# Autodesk Inventor assembly: Shooter
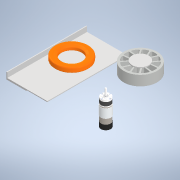
[picture p0: Inventor's stored thumbnail of the model, 180x180]
Saved by Autodesk Inventor 2021 (Build 250183000, 183)
## iProperties
Created: 2020-09-12
Part Number: Shooter
Document SubType Name: Assembly
Designer: deli
Author: deli
## Documents named in this file (7)
- C:\Users\deli\OneDrive - Eastside Preparatory School\FTC\Ultamite Goal\Shooter 9-12-2020.iam
- C:\Users\deli\OneDrive - Eastside Preparatory School\FTC\Ultamite Goal\am-4300 Ring.ipt
- C:\Users\deli\OneDrive - Eastside Preparatory School\FTC\Chassi\Cutting\Drill Patterns\ramp.ipt
- C:\Users\deli\OneDrive - Eastside Preparatory School\FTC\Chassi\Cutting\Drill Patterns\shootingGuide.ipt
- C:\Users\deli\OneDrive - Eastside Preparatory School\FTC\Ultamite Goal\5_ Straight Flex Wheel (30A) (217-6453).ipt
- C:\Users\deli\OneDrive - Eastside Preparatory School\FTC\Ultamite Goal\5inCompliantWheelHub.ipt
- C:\Users\deli\OneDrive - Eastside Preparatory School\FTC\Ultamite Goal\am-3461a NeveRest 4 with Motor REV3.ipt
## Components (6 placed, 6 different names)
1. am-4300 Ring:1 — Mate:3, Mate:4
2. ramp:1 — Mate:1, Mate:2, Flush:1, Mate:4
3. shootingGuide:1 — Mate:1, Mate:2, Flush:1, Mate:3
4. 5_ Straight Flex Wheel (30A) (217-6453):1 — Mate:5
5. 5inCompliantWheelHub:1 — Mate:5
6. am-3461a NeveRest 4 with Motor REV3:1
## Relationships (6: Mate 5, Flush 1)
- Mate:1: ramp:1 ↔ shootingGuide:1
- Mate:2: ramp:1 ↔ shootingGuide:1
- Flush:1: ramp:1 ↔ shootingGuide:1
- Mate:3 (63.5 mm): am-4300 Ring:1 ↔ shootingGuide:1
- Mate:4: am-4300 Ring:1 ↔ ramp:1
- Mate:5: 5_ Straight Flex Wheel (30A) (217-6453):1 ↔ 5inCompliantWheelHub:1
